# Autodesk Inventor assembly: cam-flying
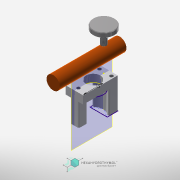
[picture p0: Inventor's stored thumbnail of the model, 180x180]
Saved by Autodesk Inventor 2016 (Build 200138000, 138)
## iProperties
Created: 2015-05-15
Part Number: cam-flying
Document SubType Name: Assembly
Designer: as
Mass: 19.8381 g
Surface Area: 51.6496 cm^2
Volume: 7.70557 cm^3
Density: 2.57451 g/cm^3
Author: as
## Documents named in this file (4)
- C:\Users\as\Documents\Inventor\mintplacer-export\cam-flying.iam
- C:\Users\as\Documents\Inventor\mintplacer-export\flying-cam-10mm.ipt
- C:\Users\as\Documents\Inventor\mintplacer-export\LibrariesContent Center Files\en-US\DIN 653\DIN 653 - M4 x 10.ipt
- C:\Users\as\Documents\Inventor\mintplacer-export\cam-flying-mount-rev2.ipt
## Components (3 placed, 3 different names)
1. cam-flying-mount-rev2:1 — Mate:2, Angle:1, Flush:1
2. flying-cam-10mm:1 — Flush:1
3. DIN 653 M4 x 10:1
## Relationships (3: Mate 1, Angle 1, Flush 1)
- Mate:2: cam-flying-mount-rev2:1
- Angle:1 (0 deg): cam-flying-mount-rev2:1
- Flush:1 (-8 mm): cam-flying-mount-rev2:1 ↔ flying-cam-10mm:1
